# Autodesk Inventor assembly: 00Assembly11
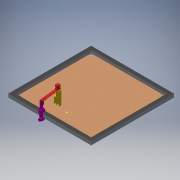
[picture p0: Inventor's stored thumbnail of the model, 180x180]
Saved by Autodesk Inventor 2019 (Build 230136000, 136)
## iProperties
Created: 2020-03-06
Part Number: 00Assembly11
Document SubType Name: Assembly
Designer: unusualgamer
Author: unusualgamer
## Documents named in this file (12)
- D:\New Folder\final.iam
- D:\assemble\Workgroups\NotInProject\strikkkk.ipt
- D:\assemble\Workgroups\NotInProject\case.ipt
- D:\assemble\Workgroups\NotInProject\M1173041- NEMA 17 (2).ipt
- D:\assemble\Workgroups\NotInProject\Part6dc.ipt
- D:\assemble\Workgroups\NotInProject\blde.ipt
- C:\Users\unusualgamer\Downloads\wheeel.0002.ipt
- D:\assemble\Workgroups\NotInProject\lclampPart3.ipt
- C:\Users\unusualgamer\Downloads\finalnut.ipt
- C:\Users\unusualgamer\Downloads\finalbolt.ipt
- D:\assemble\Workgroups\NotInProject\Part3.ipt
- D:\assemble\Workgroups\NotInProject\Part4.ipt
## Components (24 placed, 11 different names)
1. strikkkk:1 — Insert:1, Rigid:1, Rotational:10
2. case:1 — Insert:1, Insert:2, Rotational:7
3. M1173041- NEMA 17 (2):1 — Insert:2
4. Part6dc:1 — Rigid:1, Rigid:2
5. blde:1 — Rigid:2, Rotational:19
6. Part6dc:2 — Rigid:3, Rotational:21
7. Part6dc:3 — Rigid:4, Rotational:22
8. wheeel.0002:1 — Rigid:3
9. wheeel.0002:2 — Rigid:4
10. lclampPart3:1 — Rotational:3, Rotational:6, Rotational:7, Rotational:8, Rotational:9, Rotational:12, Rotational:13, Rotational:14
11. finalnut:1 — Rotational:3, Rotational:16
12. finalnut:3 — Rotational:6, Rotational:14, Rotational:15, Rotational:23
13. finalnut:4 — Rotational:9, Rotational:12, Rotational:17
14. finalnut:6 — Rotational:8, Rotational:13, Rotational:18
15. finalnut:7 — Rotational:10, Rotational:11
16. finalbolt:1 — Rotational:11
17. finalbolt:2 — Rotational:16
18. finalbolt:3 — Rotational:15
19. finalbolt:4 — Rotational:17
20. finalbolt:5 — Rotational:18
21. finalnut:8 — Rotational:19, Rotational:20
22. finalbolt:6 — Rotational:20
23. Part3:1 — Rotational:21, Rotational:22, Rotational:23
24. Part4:1
## Relationships (25: RevoluteJoint 19, WeldJoint 4, Insert 2)
- Insert:1: strikkkk:1 ↔ case:1
- Insert:2 (-22.86 mm): case:1 ↔ M1173041- NEMA 17 (2):1
- Rigid:1 [WeldJoint] (13 mm): strikkkk:1 ↔ Part6dc:1
- Rigid:2 [WeldJoint] (-5.08 mm): Part6dc:1 ↔ blde:1
- Rigid:3 [WeldJoint] (12.7 mm): Part6dc:2 ↔ wheeel.0002:1
- Rigid:4 [WeldJoint] (12.7 mm): Part6dc:3 ↔ wheeel.0002:2
- Rotational:3 [RevoluteJoint] (10.16 mm): lclampPart3:1 ↔ finalnut:1
- Rotational:6 [RevoluteJoint] (10.16 mm): lclampPart3:1 ↔ finalnut:3
- Rotational:7 [RevoluteJoint]: case:1 ↔ lclampPart3:1
- Rotational:8 [RevoluteJoint] (10.16 mm): lclampPart3:1 ↔ finalnut:6
- Rotational:9 [RevoluteJoint] (10.16 mm): lclampPart3:1 ↔ finalnut:4
- Rotational:10 [RevoluteJoint] (12.7 mm): strikkkk:1 ↔ finalnut:7
- Rotational:11 [RevoluteJoint]: finalnut:7 ↔ finalbolt:1
- Rotational:12 [RevoluteJoint] (12.7 mm): lclampPart3:1 ↔ finalnut:4
- Rotational:13 [RevoluteJoint] (12.192 mm): lclampPart3:1 ↔ finalnut:6
- Rotational:14 [RevoluteJoint] (-11.43 mm): lclampPart3:1 ↔ finalnut:3
- Rotational:15 [RevoluteJoint] (-3.81 mm): finalnut:3 ↔ finalbolt:3
- Rotational:16 [RevoluteJoint] (-3.81 mm): finalnut:1 ↔ finalbolt:2
- Rotational:17 [RevoluteJoint] (-3.81 mm): finalnut:4 ↔ finalbolt:4
- Rotational:18 [RevoluteJoint] (-3.81 mm): finalnut:6 ↔ finalbolt:5
- Rotational:19 [RevoluteJoint] (10.16 mm): blde:1 ↔ finalnut:8
- Rotational:20 [RevoluteJoint]: finalnut:8 ↔ finalbolt:6
- Rotational:21 [RevoluteJoint]: Part6dc:2 ↔ Part3:1
- Rotational:22 [RevoluteJoint]: Part6dc:3 ↔ Part3:1
- Rotational:23 [RevoluteJoint]: finalnut:3 ↔ Part3:1
